# Autodesk Inventor assembly: Ensamblaje_final2
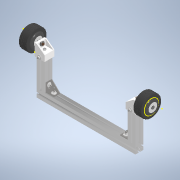
[picture p0: Inventor's stored thumbnail of the model, 180x180]
Saved by Autodesk Inventor 2021 (Build 250183000, 183)
## iProperties
Created: 2020-11-09
Part Number: Ensamblaje_final2
Document SubType Name: Assembly
Designer: juanm
Author: juanm
## Documents named in this file (22)
- C:\Users\juanm\OneDrive\Documentos\Inventor\NombreProyecto\Ensamblaje_final2.iam
- C:\Users\juanm\OneDrive\Documentos\Inventor\NombreProyecto\Horizontal.ipt
- C:\Users\juanm\OneDrive\Documentos\Inventor\NombreProyecto\Vertical.ipt
- C:\Users\juanm\OneDrive\Documentos\Inventor\NombreProyecto\Tornillo.ipt
- C:\Users\juanm\OneDrive\Documentos\Inventor\NombreProyecto\Sujetador2.ipt
- C:\Users\juanm\OneDrive\Documentos\Inventor\NombreProyecto\Tuerca para tornillo.ipt
- C:\Users\juanm\OneDrive\Documentos\Inventor\NombreProyecto\Llanta.ipt
- C:\Users\juanm\OneDrive\Documentos\Inventor\NombreProyecto\Socket.ipt
- C:\Users\juanm\OneDrive\Documentos\Inventor\NombreProyecto\Rondana.ipt
- C:\Users\juanm\OneDrive\Documentos\Inventor\NombreProyecto\TuercaLlanta.ipt
- C:\Users\juanm\OneDrive\Documentos\Inventor\NombreProyecto\UnionLlantaOmega2.ipt
- C:\Users\juanm\OneDrive\Documentos\Inventor\NombreProyecto\Tornillo_MIR.ipt
- C:\Users\juanm\OneDrive\Documentos\Inventor\NombreProyecto\Tuerca para tornillo_MIR.ipt
- C:\Users\juanm\OneDrive\Documentos\Inventor\NombreProyecto\Llanta_MIR1.ipt
- C:\Users\juanm\OneDrive\Documentos\Inventor\NombreProyecto\UnionLlantaOmega2_MIR.ipt
- C:\Users\juanm\OneDrive\Documentos\Inventor\NombreProyecto\Tornillo_MIR1.ipt
- C:\Users\juanm\OneDrive\Documentos\Inventor\NombreProyecto\Rondana_MIR2.ipt
- C:\Users\juanm\OneDrive\Documentos\Inventor\NombreProyecto\TuercaLlanta_MIR1.ipt
- C:\Users\juanm\OneDrive\Documentos\Inventor\NombreProyecto\Socket_MIR2.ipt
- C:\Users\juanm\OneDrive\Documentos\Inventor\NombreProyecto\Tuerca para tornillo_MIR1.ipt
- C:\Users\juanm\OneDrive\Documentos\Inventor\NombreProyecto\Tornillo_MIR_MIR.ipt
- C:\Users\juanm\OneDrive\Documentos\Inventor\NombreProyecto\Tuerca para tornillo_MIR_MIR.ipt
## Components (31 placed, 21 different names)
1. Horizontal:1 — Nivelación:1, Nivelación:2, Coincidencia:1, Coincidencia:5, Coincidencia:7, Nivelación:3, Coincidencia:8, Coincidencia:9, Coincidencia:11, Nivelación:4, Nivelación:5, Coincidencia:15, Coincidencia:16, Coincidencia:18, Coincidencia:20, Nivelación:6, Coincidencia:35, Coincidencia:36, Coincidencia:37, Coincidencia:38, Coincidencia:39
2. Vertical:2 — Nivelación:1, Nivelación:2, Coincidencia:1, Coincidencia:3, Coincidencia:4, Coincidencia:6, Coincidencia:10, Nivelación:7, Coincidencia:40, Nivelación:8, Coincidencia:41, Coincidencia:42, Coincidencia:43
3. Tornillo:1 — Coincidencia:8, Coincidencia:9, Coincidencia:10, De rotación:2
4. Tornillo:2 — Coincidencia:3, Coincidencia:4, Coincidencia:5, De rotación:1
5. Sujetador2:1 — Coincidencia:6, Coincidencia:7, Nivelación:3
6. Tuerca para tornillo:1 — De rotación:2
7. Tuerca para tornillo:2 — De rotación:1
8. Vertical:3 — Coincidencia:11, Nivelación:4, Nivelación:5, Coincidencia:13, Coincidencia:14, Coincidencia:19, Coincidencia:21
9. Sujetador2:2 — Coincidencia:20, Coincidencia:21, Nivelación:6
10. Tornillo:3 — Coincidencia:13, Coincidencia:14, Coincidencia:15, De rotación:4
11. Tornillo:4 — Coincidencia:16, Coincidencia:18, Coincidencia:19, De rotación:3
12. Tuerca para tornillo:3 — De rotación:3
13. Tuerca para tornillo:4 — De rotación:4
14. Llanta:1 — De rotación:5, De rotación:6, De rotación:7
15. UnionLlantaOmega2:1 — Nivelación:7, Coincidencia:40, Nivelación:8, De rotación:5, De rotación:8, Coincidencia:44, Coincidencia:45, Coincidencia:46, Coincidencia:47, Coincidencia:48, Coincidencia:49
16. Tornillo:6 — Coincidencia:41, Coincidencia:42, Coincidencia:43, De rotación:9
17. Rondana:1 — De rotación:6
18. TuercaLlanta:1 — De rotación:7
19. Socket:1 — De rotación:8
20. Tuerca para tornillo:5 — De rotación:9
21. Tornillo_MIR:1 — De rotación:10
22. Tuerca para tornillo_MIR:1 — De rotación:10
23. Llanta_MIR1:1 — De rotación:11, De rotación:12, De rotación:13
24. UnionLlantaOmega2_MIR:1 — Coincidencia:50, Coincidencia:51, Coincidencia:52, Coincidencia:53, Coincidencia:54, Coincidencia:55, De rotación:11, De rotación:14
25. Tornillo_MIR1:1 — De rotación:15
26. Rondana_MIR2:1 — De rotación:12
27. TuercaLlanta_MIR1:1 — De rotación:13
28. Socket_MIR2:1 — De rotación:14
29. Tuerca para tornillo_MIR1:1 — De rotación:15
30. Tornillo_MIR_MIR:1 — De rotación:16
31. Tuerca para tornillo_MIR_MIR:1 — De rotación:16
## Relationships (63: Mate 39, RevoluteJoint 16, Flush 8)
- Nivelación:1 [Flush]: Horizontal:1 ↔ Vertical:2
- Nivelación:2 [Flush]: Horizontal:1 ↔ Vertical:2
- Coincidencia:1 [Mate]: Horizontal:1 ↔ Vertical:2
- Coincidencia:3 [Mate]: Vertical:2 ↔ Tornillo:2
- Coincidencia:4 [Mate] (2.3 mm): Vertical:2 ↔ Tornillo:2
- Coincidencia:5 [Mate] (24 mm): Horizontal:1 ↔ Tornillo:2
- Coincidencia:6 [Mate]: Vertical:2 ↔ Sujetador2:1
- Coincidencia:7 [Mate]: Horizontal:1 ↔ Sujetador2:1
- Nivelación:3 [Flush] (5 mm): Horizontal:1 ↔ Sujetador2:1
- Coincidencia:8 [Mate]: Horizontal:1 ↔ Tornillo:1
- Coincidencia:9 [Mate] (2.3 mm): Horizontal:1 ↔ Tornillo:1
- Coincidencia:10 [Mate] (24 mm): Vertical:2 ↔ Tornillo:1
- De rotación:1 [RevoluteJoint] (7 mm): Tornillo:2 ↔ Tuerca para tornillo:2
- De rotación:2 [RevoluteJoint] (-7 mm): Tornillo:1 ↔ Tuerca para tornillo:1
- Coincidencia:11 [Mate]: Horizontal:1 ↔ Vertical:3
- Nivelación:4 [Flush]: Horizontal:1 ↔ Vertical:3
- Nivelación:5 [Flush]: Horizontal:1 ↔ Vertical:3
- Coincidencia:13 [Mate]: Vertical:3 ↔ Tornillo:3
- Coincidencia:14 [Mate] (2.3 mm): Vertical:3 ↔ Tornillo:3
- Coincidencia:15 [Mate] (24 mm): Horizontal:1 ↔ Tornillo:3
- Coincidencia:16 [Mate]: Horizontal:1 ↔ Tornillo:4
- Coincidencia:18 [Mate] (2.3 mm): Horizontal:1 ↔ Tornillo:4
- Coincidencia:19 [Mate] (24 mm): Vertical:3 ↔ Tornillo:4
- Coincidencia:20 [Mate]: Horizontal:1 ↔ Sujetador2:2
- Coincidencia:21 [Mate]: Vertical:3 ↔ Sujetador2:2
- Nivelación:6 [Flush] (5 mm): Horizontal:1 ↔ Sujetador2:2
- De rotación:3 [RevoluteJoint] (-15 mm): Tornillo:4 ↔ Tuerca para tornillo:3
- De rotación:4 [RevoluteJoint] (15 mm): Tornillo:3 ↔ Tuerca para tornillo:4
- Coincidencia:35 [Mate]: Horizontal:1
- Coincidencia:36 [Mate]: Horizontal:1
- Coincidencia:37 [Mate]: Horizontal:1
- Coincidencia:38 [Mate]: Horizontal:1
- Coincidencia:39 [Mate]: Horizontal:1
- Nivelación:7 [Flush] (-5 mm): Vertical:2 ↔ UnionLlantaOmega2:1
- Coincidencia:40 [Mate]: Vertical:2 ↔ UnionLlantaOmega2:1
- Nivelación:8 [Flush] (5 mm): Vertical:2 ↔ UnionLlantaOmega2:1
- Coincidencia:41 [Mate] (-14 mm): Vertical:2 ↔ Tornillo:6
- Coincidencia:42 [Mate] (2.3 mm): Vertical:2 ↔ Tornillo:6
- Coincidencia:43 [Mate]: Vertical:2 ↔ Tornillo:6
- De rotación:5 [RevoluteJoint] (-10 mm): Llanta:1 ↔ UnionLlantaOmega2:1
- De rotación:6 [RevoluteJoint] (-22.5 mm): Llanta:1 ↔ Rondana:1
- De rotación:7 [RevoluteJoint] (-10 mm): Llanta:1 ↔ TuercaLlanta:1
- De rotación:8 [RevoluteJoint] (16 mm): UnionLlantaOmega2:1 ↔ Socket:1
- De rotación:9 [RevoluteJoint] (4.5 mm): Tornillo:6 ↔ Tuerca para tornillo:5
- Coincidencia:44 [Mate]: UnionLlantaOmega2:1
- Coincidencia:45 [Mate]: UnionLlantaOmega2:1
- Coincidencia:46 [Mate]: UnionLlantaOmega2:1
- Coincidencia:47 [Mate]: UnionLlantaOmega2:1
- Coincidencia:48 [Mate]: UnionLlantaOmega2:1
- Coincidencia:49 [Mate]: UnionLlantaOmega2:1
- De rotación:10 [RevoluteJoint] (-4.5 mm): Tornillo_MIR:1 ↔ Tuerca para tornillo_MIR:1
- Coincidencia:50 [Mate]: UnionLlantaOmega2_MIR:1
- Coincidencia:51 [Mate]: UnionLlantaOmega2_MIR:1
- Coincidencia:52 [Mate]: UnionLlantaOmega2_MIR:1
- Coincidencia:53 [Mate]: UnionLlantaOmega2_MIR:1
- Coincidencia:54 [Mate]: UnionLlantaOmega2_MIR:1
- Coincidencia:55 [Mate]: UnionLlantaOmega2_MIR:1
- De rotación:11 [RevoluteJoint] (10 mm): Llanta_MIR1:1 ↔ UnionLlantaOmega2_MIR:1
- De rotación:12 [RevoluteJoint] (22.5 mm): Llanta_MIR1:1 ↔ Rondana_MIR2:1
- De rotación:13 [RevoluteJoint] (10 mm): Llanta_MIR1:1 ↔ TuercaLlanta_MIR1:1
- De rotación:14 [RevoluteJoint] (-16 mm): UnionLlantaOmega2_MIR:1 ↔ Socket_MIR2:1
- De rotación:15 [RevoluteJoint] (-4.5 mm): Tornillo_MIR1:1 ↔ Tuerca para tornillo_MIR1:1
- De rotación:16 [RevoluteJoint] (4.5 mm): Tornillo_MIR_MIR:1 ↔ Tuerca para tornillo_MIR_MIR:1
